# Autodesk Inventor assembly: UPPER_LEG_ASM
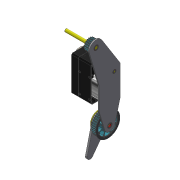
[picture p0: Inventor's stored thumbnail of the model, 180x180]
Saved by Autodesk Inventor 2019.4 (Build 234330000, 330)
## iProperties
Created: 2019-11-12
Part Number: UPPER_LEG_ASM
Material: 一般
Document SubType Name: Assembly
Designer: y6tada
Author: y6tada
## Documents named in this file (7)
- C:\Workspace\Yuni9\Inventor\Asm\UPPER_LEG\UPPER_LEG_ASM.iam
- C:\Workspace\Yuni9\Inventor\Libs\DYNAMIXEL\XM540\XM540_NO_BACK.iam
- C:\Workspace\Yuni9\Inventor\Asm\UPPER_LEG\ANKLE_DRIVER_LOD.ipt
- C:\Workspace\Yuni9\Inventor\Asm\UPPER_LEG\BELT_SUPPORT_INNER.iam
- C:\Workspace\Yuni9\Inventor\Asm\UPPER_LEG\KNEE_DRIVER_ASM.iam
- C:\Workspace\Yuni9\Inventor\Asm\UPPER_LEG\UPPER_LEG_OUTER_FRAME.ipt
- C:\Workspace\Yuni9\Inventor\Asm\UPPER_LEG\COXA_PITCH_DRIVER_PULLEY.iam
## Components (6 placed, 6 different names)
1. XM540_NO_BACK:1 [sub-assembly] — フラッシュ:2, フラッシュ:3, メイト:31
2. ANKLE_DRIVER_LOD:1 — メイト:3
3. BELT_SUPPORT_INNER:1 [sub-assembly] — メイト:34, メイト:35
4. KNEE_DRIVER_ASM:1 [sub-assembly] — メイト:29, メイト:33
5. UPPER_LEG_OUTER_FRAME:1 — メイト:27, メイト:29, フラッシュ:2, メイト:33, メイト:34, フラッシュ:4, メイト:35
6. COXA_PITCH_DRIVER_PULLEY:1 [sub-assembly]
## Relationships (15: Mate 12, Flush 3)
- [Mate]: COXA_PITCH_DRIVER_PULLEY:1
- メイト:3 [Mate]: ANKLE_DRIVER_LOD:1
- [Mate]: COXA_PITCH_DRIVER_PULLEY:1
- [Mate] (1 mm): ANKLE_DRIVER_LOD:1 ↔ COXA_PITCH_DRIVER_PULLEY:1
- メイト:27 [Mate]: UPPER_LEG_OUTER_FRAME:1
- [Mate]: UPPER_LEG_OUTER_FRAME:1 ↔ COXA_PITCH_DRIVER_PULLEY:1
- メイト:29 [Mate]: KNEE_DRIVER_ASM:1 ↔ UPPER_LEG_OUTER_FRAME:1
- フラッシュ:2 [Flush] (-45 mm): XM540_NO_BACK:1 ↔ UPPER_LEG_OUTER_FRAME:1
- フラッシュ:3 [Flush] (75 mm): XM540_NO_BACK:1
- メイト:31 [Mate]: XM540_NO_BACK:1
- [Mate]: COXA_PITCH_DRIVER_PULLEY:1
- メイト:33 [Mate]: KNEE_DRIVER_ASM:1 ↔ UPPER_LEG_OUTER_FRAME:1
- メイト:34 [Mate]: BELT_SUPPORT_INNER:1 ↔ UPPER_LEG_OUTER_FRAME:1
- フラッシュ:4 [Flush]: UPPER_LEG_OUTER_FRAME:1
- メイト:35 [Mate]: BELT_SUPPORT_INNER:1 ↔ UPPER_LEG_OUTER_FRAME:1
